# Autodesk Inventor assembly: Assembly_Cube_empty_1x1_v2
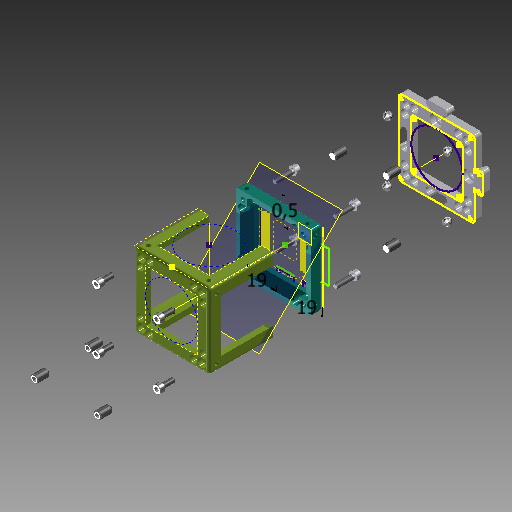
[picture p0: Inventor's stored thumbnail of the model, 512x512]
Saved by Autodesk Inventor 2019 (Build 230136000, 136)
## iProperties
Created: 2018-06-11
Part Number: Assembly_Cube_empty_1x1_v2
Material: Generisch
Document SubType Name: Assembly
Designer: diederichbenedict
Mass: 28.3962 g
Surface Area: 161.576 cm^2
Volume: 24.38 cm^3
Density: 1.16473 g/cm^3
Author: diederichbenedict
## Documents named in this file (8)
- C:\Users\UC2\Dropbox\UC2\02_CAD\INVENTOR\uc2_v3\Assembly_Cube_explosion_1x1_v3.iam
- C:\Users\UC2\Dropbox\UC2\02_CAD\INVENTOR\uc2_v3\10_Cube_1x1_v3.ipt
- C:\Users\UC2\Dropbox\UC2\02_CAD\INVENTOR\uc2_v3\10_Lid_1x1_v3.ipt
- C:\Users\UC2\Documents\Inventor\Content Center Files\R2019\de-DE\DIN 912\DIN 912 - M3 x 0,5 x 12 x 10,75.ipt
- C:\Users\UC2\Documents\Inventor\Content Center Files\R2019\de-DE\DIN 912\DIN 912 - M3 x 0,5 x 8 x 6,75.ipt
- C:\Users\UC2\Dropbox\UC2\02_CAD\INVENTOR\uc2_v3\10_Base_puzzle_v3.ipt
- C:\Users\UC2\Documents\Inventor\Content Center Files\R2019\de-DE\ISO 4026\ISO 4026 - M5 x 8 - ISO.ipt
- C:\Users\UC2\Dropbox\UC2\02_CAD\INVENTOR\uc2_v3\00_BallMagnets_5mm.ipt
## Components (18 placed, 7 different names)
1. 10_Cube_1x1_v3:1 — Mate:3, Mate:2, Angle:3, Mate:4, Mate:5, Mate:6, Mate:7, Flush:9
2. 10_Lid_1x1_v3:1 — Mate:3, Mate:2, Flush:3, Flush:4, Flush:5, Angle:3, Mate:14, Angle:4, Mate:15, Mate:16, Mate:17, Mate:18, Mate:19, Flush:19
3. DIN 912 - ersetzt durch DIN EN ISO 4762 M3 x 12:5 — Mate:18, Flush:17
4. DIN 912 - ersetzt durch DIN EN ISO 4762 M3 x 12:6 — Mate:16, Flush:16, Flush:17, Flush:18, Flush:19
5. DIN 912 - ersetzt durch DIN EN ISO 4762 M3 x 12:7 — Mate:19, Flush:16
6. DIN 912 - ersetzt durch DIN EN ISO 4762 M3 x 12:8 — Mate:17, Flush:18
7. ISO 4026 M5 x 8:1
8. ISO 4026 M5 x 8:2
9. ISO 4026 M5 x 8:3
10. ISO 4026 M5 x 8:4
11. ISO 4026 M5 x 8:5
12. ISO 4026 M5 x 8:6
13. DIN 912 - ersetzt durch DIN EN ISO 4762 M3 x 8:1 — Mate:4, Flush:6, Flush:7, Flush:8, Flush:9
14. DIN 912 - ersetzt durch DIN EN ISO 4762 M3 x 8:2 — Mate:5, Flush:7
15. DIN 912 - ersetzt durch DIN EN ISO 4762 M3 x 8:3 — Mate:6, Flush:6
16. DIN 912 - ersetzt durch DIN EN ISO 4762 M3 x 8:4 — Mate:7, Flush:8
17. 10_Base_puzzle_v3:1 — Mate:14, Angle:4, Mate:15, Passend:20, Passend:21
18. 00_BallMagnets_5mm:1 — Passend:20, Passend:21
## Relationships (39: Mate 20, Flush 17, Angle 2)
- Mate:3 (25 mm): 10_Cube_1x1_v3:1 ↔ 10_Lid_1x1_v3:1
- Mate:2: 10_Cube_1x1_v3:1 ↔ 10_Lid_1x1_v3:1
- Flush:3: 10_Lid_1x1_v3:1
- Flush:4: 10_Lid_1x1_v3:1
- Flush:5: 10_Lid_1x1_v3:1
- Angle:3 (0 deg): 10_Cube_1x1_v3:1 ↔ 10_Lid_1x1_v3:1
- Mate:4: 10_Cube_1x1_v3:1 ↔ DIN 912 - ersetzt durch DIN EN ISO 4762 M3 x 8:1
- Mate:5: 10_Cube_1x1_v3:1 ↔ DIN 912 - ersetzt durch DIN EN ISO 4762 M3 x 8:2
- Mate:6: 10_Cube_1x1_v3:1 ↔ DIN 912 - ersetzt durch DIN EN ISO 4762 M3 x 8:3
- Mate:7: 10_Cube_1x1_v3:1 ↔ DIN 912 - ersetzt durch DIN EN ISO 4762 M3 x 8:4
- Flush:6: DIN 912 - ersetzt durch DIN EN ISO 4762 M3 x 8:1 ↔ DIN 912 - ersetzt durch DIN EN ISO 4762 M3 x 8:3
- Flush:7: DIN 912 - ersetzt durch DIN EN ISO 4762 M3 x 8:1 ↔ DIN 912 - ersetzt durch DIN EN ISO 4762 M3 x 8:2
- Flush:8: DIN 912 - ersetzt durch DIN EN ISO 4762 M3 x 8:1 ↔ DIN 912 - ersetzt durch DIN EN ISO 4762 M3 x 8:4
- Flush:9 (-30 mm): 10_Cube_1x1_v3:1 ↔ DIN 912 - ersetzt durch DIN EN ISO 4762 M3 x 8:1
- [Mate]: 10_Cube_1x1_v3:1 ↔ ISO 4026 M5 x 8:1
- [Mate]: 10_Cube_1x1_v3:1 ↔ ISO 4026 M5 x 8:2
- [Mate]: 10_Cube_1x1_v3:1 ↔ ISO 4026 M5 x 8:3
- [Flush]: ISO 4026 M5 x 8:1 ↔ ISO 4026 M5 x 8:2
- [Flush]: ISO 4026 M5 x 8:1 ↔ ISO 4026 M5 x 8:3
- [Flush] (-70 mm): 10_Cube_1x1_v3:1 ↔ ISO 4026 M5 x 8:1
- [Mate]: 10_Lid_1x1_v3:1 ↔ ISO 4026 M5 x 8:5
- [Mate]: 10_Lid_1x1_v3:1 ↔ ISO 4026 M5 x 8:6
- [Mate]: 10_Lid_1x1_v3:1 ↔ ISO 4026 M5 x 8:4
- [Flush]: ISO 4026 M5 x 8:4 ↔ ISO 4026 M5 x 8:6
- [Flush]: ISO 4026 M5 x 8:5 ↔ ISO 4026 M5 x 8:6
- [Flush] (-60 mm): 10_Lid_1x1_v3:1 ↔ ISO 4026 M5 x 8:6
- Mate:14: 10_Lid_1x1_v3:1 ↔ 10_Base_puzzle_v3:1
- Angle:4 (0 deg): 10_Lid_1x1_v3:1 ↔ 10_Base_puzzle_v3:1
- Mate:15 (100 mm): 10_Lid_1x1_v3:1 ↔ 10_Base_puzzle_v3:1
- Mate:16: 10_Lid_1x1_v3:1 ↔ DIN 912 - ersetzt durch DIN EN ISO 4762 M3 x 12:6
- Mate:17: 10_Lid_1x1_v3:1 ↔ DIN 912 - ersetzt durch DIN EN ISO 4762 M3 x 12:8
- Mate:18: 10_Lid_1x1_v3:1 ↔ DIN 912 - ersetzt durch DIN EN ISO 4762 M3 x 12:5
- Mate:19: 10_Lid_1x1_v3:1 ↔ DIN 912 - ersetzt durch DIN EN ISO 4762 M3 x 12:7
- Flush:16: DIN 912 - ersetzt durch DIN EN ISO 4762 M3 x 12:6 ↔ DIN 912 - ersetzt durch DIN EN ISO 4762 M3 x 12:7
- Flush:17: DIN 912 - ersetzt durch DIN EN ISO 4762 M3 x 12:5 ↔ DIN 912 - ersetzt durch DIN EN ISO 4762 M3 x 12:6
- Flush:18: DIN 912 - ersetzt durch DIN EN ISO 4762 M3 x 12:6 ↔ DIN 912 - ersetzt durch DIN EN ISO 4762 M3 x 12:8
- Flush:19 (-28 mm): 10_Lid_1x1_v3:1 ↔ DIN 912 - ersetzt durch DIN EN ISO 4762 M3 x 12:6
- Passend:20 [Mate]: 10_Base_puzzle_v3:1 ↔ 00_BallMagnets_5mm:1
- Passend:21 [Mate]: 10_Base_puzzle_v3:1 ↔ 00_BallMagnets_5mm:1
